# Autodesk Inventor assembly: .HingeMK2
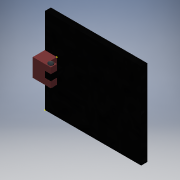
[picture p0: Inventor's stored thumbnail of the model, 180x180]
Saved by Autodesk Inventor 2016 (Build 200138000, 138)
## iProperties
Created: 2017-02-18
Part Number: .HingeMK2
Document SubType Name: Assembly
Designer: RoboticsUser
Author: RoboticsUser
## Documents named in this file (4)
- C:\Robotics\CAD\2016-17_CAD\.HingeMK2.iam
- C:\Robotics\CAD\2016-17_CAD\HingePart2MK2.ipt
- C:\Robotics\CAD\2016-17_CAD\HingePart1MK2.ipt
- C:\Robotics\CAD\2016-17_CAD\HingePart3MK2.ipt
## Components (3 placed, 3 different names)
1. HingePart2MK2:1 — Mate:1, Flush:1, Mate:2, Mate:3, Mate:4
2. HingePart1MK2:1 — Mate:1, Flush:1, Mate:2
3. HingePart3MK2:1 — Mate:3, Mate:4
## Relationships (5: Mate 4, Flush 1)
- Mate:1: HingePart2MK2:1 ↔ HingePart1MK2:1
- Flush:1: HingePart2MK2:1 ↔ HingePart1MK2:1
- Mate:2 (0.0762 mm): HingePart2MK2:1 ↔ HingePart1MK2:1
- Mate:3: HingePart2MK2:1 ↔ HingePart3MK2:1
- Mate:4: HingePart2MK2:1 ↔ HingePart3MK2:1
